# Autodesk Inventor assembly: Assembly base
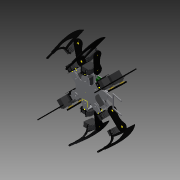
[picture p0: Inventor's stored thumbnail of the model, 180x180]
Saved by Autodesk Inventor 2015 (Build 190159000, 159)
## iProperties
Created: 2015-12-27
Part Number: Assembly base
Document SubType Name: Assembly
Designer: William
Author: William
## Documents named in this file (13)
- D:\Kuliah\Kepanitiaan\TI KRPAI Berkaki TRUI\Reva\FIXED\Assembly base.iam
- D:\Kuliah\Kepanitiaan\TI KRPAI Berkaki TRUI\Reva\BASE NEWWWW3.ipt
- D:\Kuliah\Kepanitiaan\TI KRPAI Berkaki TRUI\Reva\servo.ipt
- D:\Kuliah\Kepanitiaan\TI KRPAI Berkaki TRUI\Reva\bracket khusus.ipt
- D:\Kuliah\Kepanitiaan\TI KRPAI Berkaki TRUI\Reva\Assembly2.1.iam
- D:\Kuliah\Kepanitiaan\TI KRPAI Berkaki TRUI\Reva\Assembly2.iam
- D:\Kuliah\Kepanitiaan\TI KRPAI Berkaki TRUI\Reva\tibia servo.iam
- D:\Kuliah\Kepanitiaan\TI KRPAI Berkaki TRUI\Reva\femurpendek horn.iam
- D:\Kuliah\Kepanitiaan\TI KRPAI Berkaki TRUI\Reva\tibia servo2.iam
- D:\Kuliah\Kepanitiaan\TI KRPAI Berkaki TRUI\Reva\bayi.ipt
- D:\Kuliah\Kepanitiaan\TI KRPAI Berkaki TRUI\Reva\Spacer 5cm.ipt
- D:\Kuliah\Kepanitiaan\TI KRPAI Berkaki TRUI\Reva\ssc-32.ipt
- D:\Kuliah\Kepanitiaan\TI KRPAI Berkaki TRUI\Reva\Part3.ipt
## Components (38 placed, 12 different names)
1. BASE NEWWWW3:1 — Mate:55, Mate:56, Mate:58, Mate:59, Mate:60, Mate:61, Mate:62, Mate:63, Mate:64, Mate:65, Mate:66, Mate:70, Mate:71
2. servo:1 — Mate:11, Mate:12
3. servo:2 — Mate:3, Mate:4
4. servo:3 — Mate:1, Mate:2
5. servo:4 — Mate:5, Mate:6, Mate:55, Mate:56
6. servo:5 — Mate:7, Mate:8, Mate:58
7. servo:6 — Mate:9, Mate:10
8. bracket khusus:1 — Mate:3, Mate:4, Mate:13, Mate:14, Mate:15
9. bracket khusus:2 — Mate:1, Mate:2, Mate:16, Mate:17, Mate:18
10. bracket khusus:3 — Mate:5, Mate:6, Mate:19, Mate:20, Mate:21
11. bracket khusus:4 — Mate:7, Mate:8, Mate:28, Mate:29, Mate:30, Rotational:1
12. bracket khusus:5 — Mate:9, Mate:10, Mate:25, Mate:26, Mate:27
13. bracket khusus:6 — Mate:11, Mate:12, Mate:22, Mate:23, Mate:24
14. Assembly2.1:1 [sub-assembly] — Mate:13, Mate:14, Mate:15, Mate:31, Mate:32
15. Assembly2.1:2 [sub-assembly] — Mate:16, Mate:17, Mate:18, Mate:33, Mate:34
16. Assembly2.1:3 [sub-assembly] — Mate:19, Mate:20, Mate:21, Mate:35, Mate:36
17. Assembly2:1 [sub-assembly] — Mate:28, Mate:29, Mate:30, Mate:41, Mate:42
18. Assembly2:2 [sub-assembly] — Mate:25, Mate:26, Mate:27, Mate:39, Mate:40
19. Assembly2:3 [sub-assembly] — Mate:22, Mate:23, Mate:24, Mate:37, Mate:38
20. tibia servo:1 [sub-assembly] — Mate:43, Mate:44
21. tibia servo:2 [sub-assembly] — Mate:45, Mate:46
22. tibia servo:3 [sub-assembly] — Mate:47, Mate:48
23. femurpendek horn:1 [sub-assembly] — Mate:31, Mate:32, Mate:53, Mate:54
24. femurpendek horn:2 [sub-assembly] — Mate:33, Mate:34, Mate:51, Mate:52
25. femurpendek horn:3 [sub-assembly] — Mate:35, Mate:36, Mate:49, Mate:50
26. femurpendek horn:4 [sub-assembly] — Mate:37, Mate:38, Mate:43, Mate:44
27. femurpendek horn:5 [sub-assembly] — Mate:39, Mate:40, Mate:45, Mate:46
28. femurpendek horn:6 [sub-assembly] — Mate:41, Mate:42, Mate:47, Mate:48
29. tibia servo2:1 [sub-assembly] — Mate:49, Mate:50
30. tibia servo2:2 [sub-assembly] — Mate:51, Mate:52
31. tibia servo2:3 [sub-assembly] — Mate:53, Mate:54
32. bayi:1 — Mate:70, Mate:71
33. Spacer 5cm:1 — Mate:60, Mate:61
34. Spacer 5cm:2 — Mate:65, Mate:66, Mate:69
35. Spacer 5cm:3 — Mate:63, Mate:64
36. Spacer 5cm:4 — Mate:59, Mate:62, Mate:67
37. ssc-32:1 — Mate:67, Mate:69
38. Part3:1 — Rotational:1
## Relationships (70: Mate 69, RevoluteJoint 1)
- Mate:1: servo:3 ↔ bracket khusus:2
- Mate:2: servo:3 ↔ bracket khusus:2
- Mate:3: servo:2 ↔ bracket khusus:1
- Mate:4: servo:2 ↔ bracket khusus:1
- Mate:5: servo:4 ↔ bracket khusus:3
- Mate:6: servo:4 ↔ bracket khusus:3
- Mate:7: servo:5 ↔ bracket khusus:4
- Mate:8: servo:5 ↔ bracket khusus:4
- Mate:9: servo:6 ↔ bracket khusus:5
- Mate:10: servo:6 ↔ bracket khusus:5
- Mate:11: servo:1 ↔ bracket khusus:6
- Mate:12: servo:1 ↔ bracket khusus:6
- Mate:13: bracket khusus:1 ↔ Assembly2.1:1
- Mate:14: bracket khusus:1 ↔ Assembly2.1:1
- Mate:15: bracket khusus:1 ↔ Assembly2.1:1
- Mate:16: bracket khusus:2 ↔ Assembly2.1:2
- Mate:17: bracket khusus:2 ↔ Assembly2.1:2
- Mate:18: bracket khusus:2 ↔ Assembly2.1:2
- Mate:19: bracket khusus:3 ↔ Assembly2.1:3
- Mate:20: bracket khusus:3 ↔ Assembly2.1:3
- Mate:21: bracket khusus:3 ↔ Assembly2.1:3
- Mate:22: bracket khusus:6 ↔ Assembly2:3
- Mate:23: bracket khusus:6 ↔ Assembly2:3
- Mate:24: bracket khusus:6 ↔ Assembly2:3
- Mate:25: bracket khusus:5 ↔ Assembly2:2
- Mate:26: bracket khusus:5 ↔ Assembly2:2
- Mate:27: bracket khusus:5 ↔ Assembly2:2
- Mate:28: bracket khusus:4 ↔ Assembly2:1
- Mate:29: bracket khusus:4 ↔ Assembly2:1
- Mate:30: bracket khusus:4 ↔ Assembly2:1
- Mate:31: Assembly2.1:1 ↔ femurpendek horn:1
- Mate:32: Assembly2.1:1 ↔ femurpendek horn:1
- Mate:33: Assembly2.1:2 ↔ femurpendek horn:2
- Mate:34: Assembly2.1:2 ↔ femurpendek horn:2
- Mate:35: Assembly2.1:3 ↔ femurpendek horn:3
- Mate:36: Assembly2.1:3 ↔ femurpendek horn:3
- Mate:37: Assembly2:3 ↔ femurpendek horn:4
- Mate:38: Assembly2:3 ↔ femurpendek horn:4
- Mate:39: Assembly2:2 ↔ femurpendek horn:5
- Mate:40: Assembly2:2 ↔ femurpendek horn:5
- Mate:41: Assembly2:1 ↔ femurpendek horn:6
- Mate:42: Assembly2:1 ↔ femurpendek horn:6
- Mate:43: tibia servo:1 ↔ femurpendek horn:4
- Mate:44: tibia servo:1 ↔ femurpendek horn:4
- Mate:45: tibia servo:2 ↔ femurpendek horn:5
- Mate:46: tibia servo:2 ↔ femurpendek horn:5
- Mate:47: tibia servo:3 ↔ femurpendek horn:6
- Mate:48: tibia servo:3 ↔ femurpendek horn:6
- Mate:49: femurpendek horn:3 ↔ tibia servo2:1
- Mate:50: femurpendek horn:3 ↔ tibia servo2:1
- Mate:51: femurpendek horn:2 ↔ tibia servo2:2
- Mate:52: femurpendek horn:2 ↔ tibia servo2:2
- Mate:53: femurpendek horn:1 ↔ tibia servo2:3
- Mate:54: femurpendek horn:1 ↔ tibia servo2:3
- Mate:55: BASE NEWWWW3:1 ↔ servo:4
- Mate:56: BASE NEWWWW3:1 ↔ servo:4
- Mate:58: BASE NEWWWW3:1 ↔ servo:5
- Mate:59: BASE NEWWWW3:1 ↔ Spacer 5cm:4
- Mate:60: BASE NEWWWW3:1 ↔ Spacer 5cm:1
- Mate:61: BASE NEWWWW3:1 ↔ Spacer 5cm:1
- Mate:62: BASE NEWWWW3:1 ↔ Spacer 5cm:4
- Mate:63: BASE NEWWWW3:1 ↔ Spacer 5cm:3
- Mate:64: BASE NEWWWW3:1 ↔ Spacer 5cm:3
- Mate:65: BASE NEWWWW3:1 ↔ Spacer 5cm:2
- Mate:66: BASE NEWWWW3:1 ↔ Spacer 5cm:2
- Mate:67: Spacer 5cm:4 ↔ ssc-32:1
- Mate:69: Spacer 5cm:2 ↔ ssc-32:1
- Mate:70: BASE NEWWWW3:1 ↔ bayi:1
- Mate:71: BASE NEWWWW3:1 ↔ bayi:1
- Rotational:1 [RevoluteJoint]: bracket khusus:4 ↔ Part3:1
